# Autodesk Inventor assembly: Claw
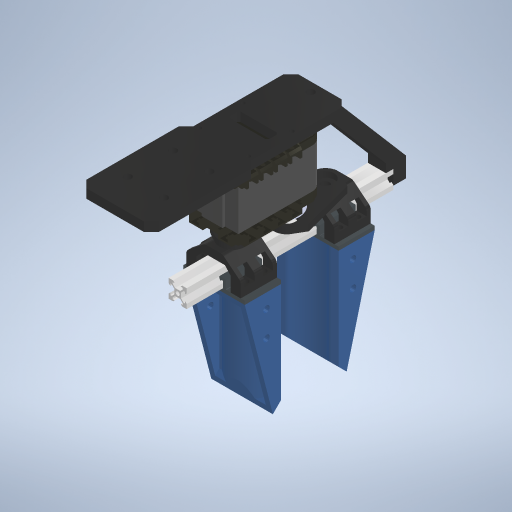
[picture p0: Inventor's stored thumbnail of the model, 512x512]
Saved by Autodesk Inventor 2024.2 (Build 282272000, 272)
## iProperties
Created: 2025-09-29
Part Number: Claw
Document SubType Name: Assembly
Designer: Admin
Author: Admin
## Documents named in this file (10)
- C:\Users\Admin\Documents\GitHub\ManipuladorCartesiano\DiseñoMecánico\Assemblies\Claw.iam
- C:\Users\Admin\Documents\GitHub\ManipuladorCartesiano\DiseñoMecánico\Assemblies\AX-12A.iam
- C:\Users\Admin\Documents\GitHub\ManipuladorCartesiano\DiseñoMecánico\AuxiliarPieces\ClawPrinted\SuperiorPiece.ipt
- C:\Users\Admin\Documents\GitHub\ManipuladorCartesiano\DiseñoMecánico\AuxiliarPieces\ClawPrinted\SoporteExterno.ipt
- C:\Users\Admin\Documents\GitHub\ManipuladorCartesiano\DiseñoMecánico\AuxiliarPieces\ClawAlPieces\Bosch1010.ipt
- C:\Users\Admin\Documents\GitHub\ManipuladorCartesiano\DiseñoMecánico\AuxiliarPieces\ClawPrinted\MechanismArm.ipt
- C:\Users\Admin\Documents\GitHub\ManipuladorCartesiano\DiseñoMecánico\AuxiliarPieces\ClawAlPieces\Axel.STEP.ipt
- C:\Users\Admin\Documents\GitHub\ManipuladorCartesiano\DiseñoMecánico\AuxiliarPieces\ClawAlPieces\SliderPiece.ipt
- C:\Users\Admin\Documents\GitHub\ManipuladorCartesiano\DiseñoMecánico\AuxiliarPieces\ClawPrinted\GripperSupport.ipt
- C:\Users\Admin\Documents\GitHub\ManipuladorCartesiano\DiseñoMecánico\AuxiliarPieces\ClawPrinted\Gripper.ipt
## Components (13 placed, 9 different names)
1. AX-12A:1 [sub-assembly] — Mate:1, Mate:2, Mate:3, Mate:8, Mate:9
2. SuperiorPiece:1 — Mate:1, Mate:2, Mate:3, Mate:4, Mate:5, Mate:6
3. SoporteExterno:1 — Mate:4, Mate:5, Mate:6, Mate:7, Flush:1, Flush:2
4. Bosch1010:1 — Mate:7, Flush:1, Flush:2, Mate:14, Mate:15, Mate:16, Mate:17
5. MechanismArm:1 — Mate:10, Mate:13, Mate:24
6. MechanismArm:2 — Mate:11, Mate:12, Mate:25
7. Axel.STEP:1 — Mate:8, Mate:9, Mate:10, Mate:11, Mate:12, Mate:13
8. SliderPiece:1 — Mate:14, Mate:15, Mate:18, Mate:19, Mate:20, Mate:29, Mate:30, Mate:31
9. SliderPiece:2 — Mate:16, Mate:17, Mate:21, Mate:22, Mate:23, Mate:26, Mate:27, Mate:28
10. GripperSupport:1 — Mate:18, Mate:19, Mate:20, Mate:25
11. GripperSupport:2 — Mate:21, Mate:22, Mate:23, Mate:24
12. Gripper:1 — Mate:26, Mate:27, Mate:28
13. Gripper:2 — Mate:29, Mate:30, Mate:31
## Relationships (33: Mate 31, Flush 2)
- Mate:1: AX-12A:1 ↔ SuperiorPiece:1
- Mate:2: AX-12A:1 ↔ SuperiorPiece:1
- Mate:3: AX-12A:1 ↔ SuperiorPiece:1
- Mate:4: SuperiorPiece:1 ↔ SoporteExterno:1
- Mate:5: SuperiorPiece:1 ↔ SoporteExterno:1
- Mate:6: SuperiorPiece:1 ↔ SoporteExterno:1
- Mate:7: SoporteExterno:1 ↔ Bosch1010:1
- Flush:1: SoporteExterno:1 ↔ Bosch1010:1
- Flush:2: SoporteExterno:1 ↔ Bosch1010:1
- Mate:8: AX-12A:1 ↔ Axel.STEP:1
- Mate:9: AX-12A:1 ↔ Axel.STEP:1
- Mate:10: MechanismArm:1 ↔ Axel.STEP:1
- Mate:11: MechanismArm:2 ↔ Axel.STEP:1
- Mate:12: MechanismArm:2 ↔ Axel.STEP:1
- Mate:13: MechanismArm:1 ↔ Axel.STEP:1
- Mate:14: Bosch1010:1 ↔ SliderPiece:1
- Mate:15: Bosch1010:1 ↔ SliderPiece:1
- Mate:16: Bosch1010:1 ↔ SliderPiece:2
- Mate:17: Bosch1010:1 ↔ SliderPiece:2
- Mate:18: SliderPiece:1 ↔ GripperSupport:1
- Mate:19: SliderPiece:1 ↔ GripperSupport:1
- Mate:20: SliderPiece:1 ↔ GripperSupport:1
- Mate:21: SliderPiece:2 ↔ GripperSupport:2
- Mate:22: SliderPiece:2 ↔ GripperSupport:2
- Mate:23: SliderPiece:2 ↔ GripperSupport:2
- Mate:24: MechanismArm:1 ↔ GripperSupport:2
- Mate:25: MechanismArm:2 ↔ GripperSupport:1
- Mate:26: SliderPiece:2 ↔ Gripper:1
- Mate:27: SliderPiece:2 ↔ Gripper:1
- Mate:28: SliderPiece:2 ↔ Gripper:1
- Mate:29: SliderPiece:1 ↔ Gripper:2
- Mate:30: SliderPiece:1 ↔ Gripper:2
- Mate:31: SliderPiece:1 ↔ Gripper:2
